# Autodesk Inventor assembly: SBGSNA6200ZZ-20
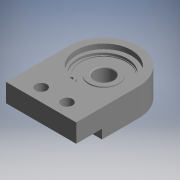
[picture p0: Inventor's stored thumbnail of the model, 180x180]
Saved by Autodesk Inventor 2017.3 (Build 213256000, 256)
## iProperties
Category: PARTsolutions
Company: MISUMI
Part Number: SBGSNA6200ZZ-20
Catalog Web Link: www.cadenas.de
Description: BGSNAB, BGSNA, SBGSNA-Bearings with Housings - Front Mount, Shouldered, h selectable/ Retained Bearing
Vendor: MISUMI
Document SubType Name: Assembly
Designer: partserver
Manufacturer: MISUMI
Mass: 20.1228 g
Surface Area: 100.175 cm^2
Volume: 20.1228 cm^3
Density: 1 g/cm^3
Title: SBGSNA6200ZZ-20
Author: Cadenas PARTsolutions
Comments: Bearings with Housings - Front Mount, Shouldered, h selectable/ Retained Bearing
PSOL_IDENT_0: {$CADENAS_DATA\23d-libs\misumi\metric\12_bearing_holders\bgsna_asmtab.prj},222 {VTYP=3D},{STYP=ASSTA
PSOL_IDENT_1: B},{NB=SBGSNA6200ZZ-20},{LINA=SBGSNA6200ZZ-20},{NN=BGSNAB, BGSNA, SBGSNA},{DATE=09.09.2019 15:26:55}
PSOL_IDENT_2: ,{GEOMDATE=23.07.2015 04:20:24},{VERSION=},{LINEID=30},{WBVAR=MATB,STH,SEAL,HH,ALT1},{WBNUMERIC=HH}
PSOL_IDENT_3: {NB=SBGSNA6200ZZ-20},{LINA=SBGSNA6200ZZ-20},{KT=DUMMY},{PN=SBGSNA6200ZZ-20},{TYPE=SBGSNA},{MATB=SST
PSOL_IDENT_4: },{MATBALG= 'ST','Steel','SST','Stainless Steel' },{STH=},{STHALG= '','-' },{ARR=304 Stainless Steel
PSOL_IDENT_5: },{ARRALG=-S},{BN=6200},{SEAL=ZZ},{SEALALG= 'ZZ','ZZ(Double Shielded)','VV','VV(Non-contact Rubber S
PSOL_IDENT_6: eal)','DD','DD(Contact Rubber Seal)' },{HH=20},{HHALG=20,25,30},{DD=10},{D=30},{DDHH=24},{B=9},{H=53
PSOL_IDENT_7: .0},{HH1=7},{L=38},{L1=14},{T=15},{T1=10},{DD1=6},{ALT1=},{ALT1ALG= '','Bearing and Retaining Ring A
PSOL_IDENT_8: ssembled','NA','with NA (Bearing and Retaining Ring not Assembled)' },{ALT1PN=},{DD3=31.4},{TT=1.20}
PSOL_IDENT_9: ,{PPATH=bgsna/bgsna_asmtpl.prj},{M=1.35}
NB: SBGSNA6200ZZ-20
NN: BGSNAB, BGSNA, SBGSNA
NT: Bearings with Housings - Front Mount, Shouldered, h selectable/ Retained Bearing
NBSYN: $PN.
LINA: SBGSNA6200ZZ-20
CATALOG: Misumi
PN: SBGSNA6200ZZ-20
MATB: Stainless Steel
STH: -
ARR: 304 Stainless Steel
BN: 6200
SEAL: ZZ(Double Shielded)
HH: 20
DD: 10
D: 30
DDHH: 24
B: 9
H: 53
HH1: 7
L: 38
L1: 14
T: 15
T1: 10
DD1: 6
ALT1: Bearing and Retaining Ring Assembled
SUPPLIER: MISUMI
ARTICLENO: SBGSNA6200ZZ-20
BOMINFO: SBGSNA6200ZZ-20
CREATOR: CADENAS GmbH
## Documents named in this file (4)
- e:\temp\worker_19\temp\exporttempdir_3676_108_kilQG\format_0\SBGSNA6200ZZ-20.iam
- e:\temp\worker_19\temp\exporttempdir_3676_108_kilQG\format_0\SBGSNA6200ZZ-20_h.ipt
- e:\temp\worker_19\temp\exporttempdir_3676_108_kilQG\format_0\bearing_6200.ipt
- e:\temp\worker_19\temp\exporttempdir_3676_108_kilQG\format_0\RRING-C-INT-S-30.ipt
## Components (3 placed, 3 different names)
1. SBGSNA6200ZZ-20_h:1 — to_bearing_XY@1 <-> center_point_XY@2, to_bearing_Z@1 <-> center_point_Z@2, to_bearing_YZ@1 <-> center_point_YZ@2, to_retaining_ring_XY@1 <-> rr_XY@3, to_retaining_ring_Z@1 <-> rr_Z@3, to_retaining_ring_YZ@1 <-> rr_YZ@3
2. bearing_6200:1 — to_bearing_XY@1 <-> center_point_XY@2, to_bearing_Z@1 <-> center_point_Z@2, to_bearing_YZ@1 <-> center_point_YZ@2
3. RRING-C-INT-S-30:1 — to_retaining_ring_XY@1 <-> rr_XY@3, to_retaining_ring_Z@1 <-> rr_Z@3, to_retaining_ring_YZ@1 <-> rr_YZ@3
## Relationships (6: Mate 4, Angle 2)
- to_bearing_XY@1 <-> center_point_XY@2 [Mate]: SBGSNA6200ZZ-20_h:1 ↔ bearing_6200:1
- to_bearing_Z@1 <-> center_point_Z@2 [Mate]: SBGSNA6200ZZ-20_h:1 ↔ bearing_6200:1
- to_bearing_YZ@1 <-> center_point_YZ@2 [Angle] (0 deg): SBGSNA6200ZZ-20_h:1 ↔ bearing_6200:1
- to_retaining_ring_XY@1 <-> rr_XY@3 [Mate]: SBGSNA6200ZZ-20_h:1 ↔ RRING-C-INT-S-30:1
- to_retaining_ring_Z@1 <-> rr_Z@3 [Mate]: SBGSNA6200ZZ-20_h:1 ↔ RRING-C-INT-S-30:1
- to_retaining_ring_YZ@1 <-> rr_YZ@3 [Angle] (0 deg): SBGSNA6200ZZ-20_h:1 ↔ RRING-C-INT-S-30:1
